# Autodesk Inventor assembly: slider-pra-gree
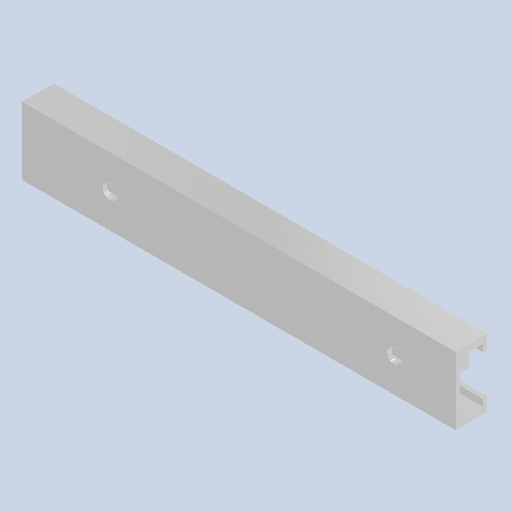
[picture p0: Inventor's stored thumbnail of the model, 512x512]
Saved by Autodesk Inventor 2024.1 (Build 281209000, 209)
## iProperties
Created: 2023-10-07
Part Number: slider-pra-gree
Document SubType Name: Assembly
Designer: haruy
Author: haruy
## Documents named in this file (3)
- C:\Users\haruy\OneDrive - Kyushu University\cad\000_parts\スライダー\slider-pra-gree.iam
- C:\Users\haruy\OneDrive - Kyushu University\cad\000_parts\スライダー\slider2a2.ipt
- C:\Users\haruy\OneDrive - Kyushu University\cad\000_parts\スライダー\slider2b.ipt
## Components (2 placed, 2 different names)
1. slider2a2:1 — メイト:1, メイト:2, メイト:3
2. slider2b:1 — メイト:1, メイト:2, メイト:3
## Relationships (3: Mate 3)
- メイト:1 [Mate]: slider2a2:1 ↔ slider2b:1
- メイト:2 [Mate]: slider2a2:1 ↔ slider2b:1
- メイト:3 [Mate]: slider2a2:1 ↔ slider2b:1
